# Autodesk Inventor assembly: MPU-9250
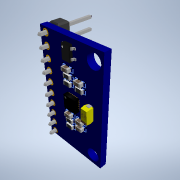
[picture p0: Inventor's stored thumbnail of the model, 180x180]
Saved by Autodesk Inventor 2020.3 (Build 243373000, 373)
## iProperties
Created: 2019-04-14
Part Number: MPU-9250
Document SubType Name: Assembly
Designer: ZEUSLAP
Author: ZEUSLAP
## Documents named in this file (9)
- C:\Users\aditk\Desktop\PETcat\withsensors\mpu-9250-9dof-imu-1.snapshot.4\MPU-9250.iam
- C:\Users\aditk\Desktop\PETcat\withsensors\mpu-9250-9dof-imu-1.snapshot.4\parts\board.ipt
- C:\Users\aditk\Desktop\PETcat\withsensors\mpu-9250-9dof-imu-1.snapshot.4\parts\hole_plating.ipt
- C:\Users\aditk\Desktop\PETcat\withsensors\mpu-9250-9dof-imu-1.snapshot.4\parts\Pin Header 1x10 TH Pitch 2.54mm.ipt
- C:\Users\aditk\Desktop\PETcat\withsensors\mpu-9250-9dof-imu-1.snapshot.4\parts\QFN-24 3x3 0.4mm.ipt
- C:\Users\aditk\Desktop\PETcat\withsensors\mpu-9250-9dof-imu-1.snapshot.4\parts\tantalum 10uF.ipt
- C:\Users\aditk\Desktop\PETcat\withsensors\mpu-9250-9dof-imu-1.snapshot.4\parts\SOT23_5.ipt
- C:\Users\aditk\Desktop\PETcat\withsensors\mpu-9250-9dof-imu-1.snapshot.4\parts\RESC-0603.ipt
- C:\Users\aditk\Desktop\PETcat\withsensors\mpu-9250-9dof-imu-1.snapshot.4\parts\CAPC-0603-T0.9-BN.ipt
## Components (35 placed, 8 different names)
1. board:1 — Mate:1, Mate:2, Mate:3, Mate:4, Mate:5, Mate:6, Mate:7, Mate:8, Mate:9, Mate:10, Mate:11, Mate:12, Mate:13, Mate:14, Mate:15, Mate:16, Mate:17, Mate:18, Mate:19, Mate:20, Mate:21, Mate:22, Mate:23, Mate:24, Mate:25, Mate:26, Mate:27, Mate:28, Mate:29, Mate:30, Mate:31, Mate:32, Mate:33, Mate:34, Mate:35, Mate:36, Mate:37, Mate:38, Mate:39, Mate:40, Mate:41, Angle:1, Angle:2, Mate:43, Flush:1, Flush:2, Mate:44, Mate:45, Angle:3, Mate:46, Mate:47, Mate:48, Angle:4, Flush:3, Flush:4, Mate:49, Mate:50, Mate:51, Mate:52, Mate:53, Mate:54, Mate:55, Mate:56, Mate:57, Mate:58, Flush:5, Flush:6, Flush:7, Flush:8, Flush:9, Flush:10, Flush:11, Flush:12, Flush:13, Flush:14, Flush:15, Flush:16, Flush:18, Flush:20, Flush:21, Mate:59, Mate:60
2. hole_plating:1 — Mate:1, Mate:2
3. hole_plating:2 — Mate:3, Mate:4
4. hole_plating:3 — Mate:13, Mate:14
5. hole_plating:4 — Mate:31, Mate:32
6. hole_plating:5 — Mate:7, Mate:8
7. hole_plating:6 — Mate:5, Mate:6
8. hole_plating:7 — Mate:9, Mate:10
9. hole_plating:8 — Mate:29, Mate:30
10. hole_plating:9 — Mate:35, Mate:36
11. hole_plating:10 — Mate:25, Mate:26
12. hole_plating:11 — Mate:19, Mate:20
13. hole_plating:12 — Mate:23, Mate:24
14. hole_plating:13 — Mate:21, Mate:22
15. hole_plating:14 — Mate:27, Mate:28
16. hole_plating:15 — Mate:33, Mate:34
17. hole_plating:16 — Mate:11, Mate:12
18. hole_plating:17 — Mate:17, Mate:18
19. hole_plating:18 — Mate:37, Mate:38
20. hole_plating:19 — Mate:15, Mate:16
21. hole_plating:20 — Mate:39, Mate:40, Mate:42
22. Pin Header 1x10 TH Pitch 2.54mm:1 — Mate:42, Angle:2, Mate:43
23. MPU-9250:1 — Mate:41, Angle:1, Flush:1, Flush:2, Mate:61
24. tantalum 10uF:1 — Mate:44, Mate:45, Angle:3, Mate:46, Mate:47, Mate:61
25. SOT23_5:1 — Mate:48, Angle:4, Flush:3, Flush:4
26. RESC-0603:1 — Mate:57, Flush:7, Flush:8
27. RESC-0603:2 — Mate:51, Flush:21, Flush:22, Flush:23
28. RESC-0603:3 — Mate:58, Flush:17, Flush:18, Flush:19, Flush:24
29. RESC-0603:4 — Mate:54, Flush:15, Flush:16, Flush:17, Flush:22
30. RESC-0603:5 — Mate:55, Flush:5, Flush:6
31. CAPC-0603-T0.9-BN:1 — Mate:49, Flush:13, Flush:14
32. CAPC-0603-T0.9-BN:2 — Mate:50, Flush:9, Flush:10
33. CAPC-0603-T0.9-BN:3 — Mate:52, Flush:19, Flush:20
34. CAPC-0603-T0.9-BN:4 — Mate:56, Flush:11, Flush:12
35. CAPC-0603-T0.9-BN:5 — Mate:53, Flush:23, Flush:24
## Relationships (89: Mate 61, Flush 24, Angle 4)
- Mate:1: board:1 ↔ hole_plating:1
- Mate:2: board:1 ↔ hole_plating:1
- Mate:3: board:1 ↔ hole_plating:2
- Mate:4: board:1 ↔ hole_plating:2
- Mate:5: board:1 ↔ hole_plating:6
- Mate:6: board:1 ↔ hole_plating:6
- Mate:7: board:1 ↔ hole_plating:5
- Mate:8: board:1 ↔ hole_plating:5
- Mate:9: board:1 ↔ hole_plating:7
- Mate:10: board:1 ↔ hole_plating:7
- Mate:11: board:1 ↔ hole_plating:16
- Mate:12: board:1 ↔ hole_plating:16
- Mate:13: board:1 ↔ hole_plating:3
- Mate:14: board:1 ↔ hole_plating:3
- Mate:15: board:1 ↔ hole_plating:19
- Mate:16: board:1 ↔ hole_plating:19
- Mate:17: board:1 ↔ hole_plating:17
- Mate:18: board:1 ↔ hole_plating:17
- Mate:19: board:1 ↔ hole_plating:11
- Mate:20: board:1 ↔ hole_plating:11
- Mate:21: board:1 ↔ hole_plating:13
- Mate:22: board:1 ↔ hole_plating:13
- Mate:23: board:1 ↔ hole_plating:12
- Mate:24: board:1 ↔ hole_plating:12
- Mate:25: board:1 ↔ hole_plating:10
- Mate:26: board:1 ↔ hole_plating:10
- Mate:27: board:1 ↔ hole_plating:14
- Mate:28: board:1 ↔ hole_plating:14
- Mate:29: board:1 ↔ hole_plating:8
- Mate:30: board:1 ↔ hole_plating:8
- Mate:31: board:1 ↔ hole_plating:4
- Mate:32: board:1 ↔ hole_plating:4
- Mate:33: board:1 ↔ hole_plating:15
- Mate:34: board:1 ↔ hole_plating:15
- Mate:35: board:1 ↔ hole_plating:9
- Mate:36: board:1 ↔ hole_plating:9
- Mate:37: board:1 ↔ hole_plating:18
- Mate:38: board:1 ↔ hole_plating:18
- Mate:39: board:1 ↔ hole_plating:20
- Mate:40: board:1 ↔ hole_plating:20
- Mate:41: board:1 ↔ MPU-9250:1
- Angle:1 (180 deg): board:1 ↔ MPU-9250:1
- Mate:42: hole_plating:20 ↔ Pin Header 1x10 TH Pitch 2.54mm:1
- Angle:2 (180 deg): board:1 ↔ Pin Header 1x10 TH Pitch 2.54mm:1
- Mate:43: board:1 ↔ Pin Header 1x10 TH Pitch 2.54mm:1
- Flush:1 (5.5 mm): board:1 ↔ MPU-9250:1
- Flush:2 (11 mm): board:1 ↔ MPU-9250:1
- Mate:44: board:1 ↔ tantalum 10uF:1
- Mate:45: board:1 ↔ tantalum 10uF:1
- Angle:3 (0 deg): board:1 ↔ tantalum 10uF:1
- Mate:46 (2 mm): board:1 ↔ tantalum 10uF:1
- Mate:47 (10.9 mm): board:1 ↔ tantalum 10uF:1
- Mate:48: board:1 ↔ SOT23_5:1
- Angle:4 (90 deg): board:1 ↔ SOT23_5:1
- Flush:3 (1 mm): board:1 ↔ SOT23_5:1
- Flush:4 (6.5 mm): board:1 ↔ SOT23_5:1
- Mate:49: board:1 ↔ CAPC-0603-T0.9-BN:1
- Mate:50: board:1 ↔ CAPC-0603-T0.9-BN:2
- Mate:51: board:1 ↔ RESC-0603:2
- Mate:52: board:1 ↔ CAPC-0603-T0.9-BN:3
- Mate:53: board:1 ↔ CAPC-0603-T0.9-BN:5
- Mate:54: board:1 ↔ RESC-0603:4
- Mate:55: board:1 ↔ RESC-0603:5
- Mate:56: board:1 ↔ CAPC-0603-T0.9-BN:4
- Mate:57: board:1 ↔ RESC-0603:1
- Mate:58: board:1 ↔ RESC-0603:3
- Flush:5 (5.5 mm): board:1 ↔ RESC-0603:5
- Flush:6 (6 mm): board:1 ↔ RESC-0603:5
- Flush:7 (7 mm): board:1 ↔ RESC-0603:1
- Flush:8 (6 mm): board:1 ↔ RESC-0603:1
- Flush:9 (6 mm): board:1 ↔ CAPC-0603-T0.9-BN:2
- Flush:10 (8.5 mm): board:1 ↔ CAPC-0603-T0.9-BN:2
- Flush:11 (9 mm): board:1 ↔ CAPC-0603-T0.9-BN:4
- Flush:12 (7 mm): board:1 ↔ CAPC-0603-T0.9-BN:4
- Flush:13 (9 mm): board:1 ↔ CAPC-0603-T0.9-BN:1
- Flush:14 (8.5 mm): board:1 ↔ CAPC-0603-T0.9-BN:1
- Flush:15 (6 mm): board:1 ↔ RESC-0603:4
- Flush:16 (8.5 mm): board:1 ↔ RESC-0603:4
- Flush:17: RESC-0603:3 ↔ RESC-0603:4
- Flush:18 (7 mm): board:1 ↔ RESC-0603:3
- Flush:19: RESC-0603:3 ↔ CAPC-0603-T0.9-BN:3
- Flush:20 (5.5 mm): board:1 ↔ CAPC-0603-T0.9-BN:3
- Flush:21 (9 mm): board:1 ↔ RESC-0603:2
- Flush:22: RESC-0603:2 ↔ RESC-0603:4
- Flush:23: RESC-0603:2 ↔ CAPC-0603-T0.9-BN:5
- Flush:24: RESC-0603:3 ↔ CAPC-0603-T0.9-BN:5
- Mate:59: board:1
- Mate:60: board:1
- Mate:61 (2.467 mm): MPU-9250:1 ↔ tantalum 10uF:1
